# Autodesk Inventor assembly: VersaPlanetary One Stage 775
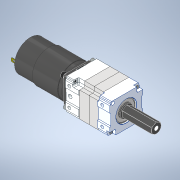
[picture p0: Inventor's stored thumbnail of the model, 180x180]
Saved by Autodesk Inventor 2022 (Build 260153000, 153)
## iProperties
Created: 2020-01-30
Part Number: VersaPlanetary One Stage 775
Document SubType Name: Assembly
Designer: aidan
Author: aidan
## Documents named in this file (10)
- C:\Users\Ty Gazaway\Documents\t3-cad\CAD\Generic and Stock\VersaPlanetary Parts\VersaPlanetary One Stage 775.iam
- C:\Users\Ty Gazaway\Documents\t3-cad\CAD\Generic and Stock\775 Pro.ipt
- C:\Users\Ty Gazaway\Documents\t3-cad\CAD\STEP Files\775_Series_Motor_Mounting_Plate.ipt
- C:\Users\Ty Gazaway\Documents\t3-cad\CAD\Generic and Stock\VersaPlanetary Parts\VersaPlanertary Mounting Block.ipt
- C:\Users\Ty Gazaway\Documents\t3-cad\CAD\Generic and Stock\VersaPlanetary Parts\VersaPlanetary Coupler.ipt
- C:\Users\Ty Gazaway\Documents\t3-cad\CAD\Generic and Stock\VersaPlanetary Parts\VersaPlanetary Motor Screw.ipt
- C:\Users\Ty Gazaway\Documents\t3-cad\CAD\Generic and Stock\VersaPlanetary Parts\VersaPlanetary Mounting Screw.ipt
- C:\Users\Ty Gazaway\Documents\t3-cad\CAD\Generic and Stock\VersaPlanetary Parts\VersaPlanetary Ring Gear.ipt
- C:\Users\Ty Gazaway\Documents\t3-cad\CAD\Generic and Stock\VersaPlanetary Parts\VersaPlanetary Long Screw.ipt
- C:\Users\Ty Gazaway\Documents\t3-cad\CAD\Generic and Stock\VersaPlanetary Parts\VersaPlanetary 0.500 Output.ipt
## Components (13 placed, 9 different names)
1. 775 Pro:1 — Mate:9, Mate:10, Mate:15, Flush:7, Mate:16, Mate:22
2. 775_Series_Motor_Mounting_Plate:1 — Mate:6, Mate:7, Mate:8, Mate:10, Mate:13, Mate:19, Flush:9
3. VersaPlanertary Mounting Block:1 — Flush:2, Mate:2, Mate:3, Mate:19, Mate:20, Mate:21, Mate:22, Flush:9, Mate:23, Mate:24, Mate:25
4. VersaPlanetary Coupler:1 — Mate:15, Flush:7
5. VersaPlanetary Motor Screw:1 — Mate:6, Flush:5, Mate:8, Mate:16
6. VersaPlanetary Motor Screw:2 — Mate:7, Flush:5, Mate:9
7. VersaPlanetary Mounting Screw:1 — Flush:6, Mate:21
8. VersaPlanetary Mounting Screw:2 — Flush:6, Mate:13, Mate:20
9. VersaPlanetary Ring Gear:1 — Flush:1, Flush:2, Flush:4, Mate:1, Mate:2, Mate:3
10. VersaPlanetary Ring Gear:2 — Flush:1, Flush:3, Flush:4, Mate:1, Mate:4, Mate:5
11. VersaPlanetary Long Screw:1 — Flush:8, Mate:25
12. VersaPlanetary Long Screw:2 — Flush:8, Mate:23, Mate:24
13. VersaPlanetary 0.500 Output:1 — Flush:3, Mate:4, Mate:5
## Relationships (29: Mate 20, Flush 9)
- Flush:1: VersaPlanetary Ring Gear:1 ↔ VersaPlanetary Ring Gear:2
- Flush:2: VersaPlanertary Mounting Block:1 ↔ VersaPlanetary Ring Gear:1
- Flush:3: VersaPlanetary Ring Gear:2 ↔ VersaPlanetary 0.500 Output:1
- Flush:4: VersaPlanetary Ring Gear:1 ↔ VersaPlanetary Ring Gear:2
- Mate:1: VersaPlanetary Ring Gear:1 ↔ VersaPlanetary Ring Gear:2
- Mate:2: VersaPlanertary Mounting Block:1 ↔ VersaPlanetary Ring Gear:1
- Mate:3: VersaPlanertary Mounting Block:1 ↔ VersaPlanetary Ring Gear:1
- Mate:4: VersaPlanetary Ring Gear:2 ↔ VersaPlanetary 0.500 Output:1
- Mate:5: VersaPlanetary Ring Gear:2 ↔ VersaPlanetary 0.500 Output:1
- Mate:6: 775_Series_Motor_Mounting_Plate:1 ↔ VersaPlanetary Motor Screw:1
- Mate:7: 775_Series_Motor_Mounting_Plate:1 ↔ VersaPlanetary Motor Screw:2
- Flush:5: VersaPlanetary Motor Screw:1 ↔ VersaPlanetary Motor Screw:2
- Mate:8: 775_Series_Motor_Mounting_Plate:1 ↔ VersaPlanetary Motor Screw:1
- Mate:9: 775 Pro:1 ↔ VersaPlanetary Motor Screw:2
- Mate:10: 775 Pro:1 ↔ 775_Series_Motor_Mounting_Plate:1
- Flush:6: VersaPlanetary Mounting Screw:1 ↔ VersaPlanetary Mounting Screw:2
- Mate:13: 775_Series_Motor_Mounting_Plate:1 ↔ VersaPlanetary Mounting Screw:2
- Mate:15: 775 Pro:1 ↔ VersaPlanetary Coupler:1
- Flush:7 (5.334 mm): 775 Pro:1 ↔ VersaPlanetary Coupler:1
- Mate:16: 775 Pro:1 ↔ VersaPlanetary Motor Screw:1
- Mate:19: 775_Series_Motor_Mounting_Plate:1 ↔ VersaPlanertary Mounting Block:1
- Flush:8: VersaPlanetary Long Screw:1 ↔ VersaPlanetary Long Screw:2
- Mate:20: VersaPlanertary Mounting Block:1 ↔ VersaPlanetary Mounting Screw:2
- Mate:21: VersaPlanertary Mounting Block:1 ↔ VersaPlanetary Mounting Screw:1
- Mate:22: 775 Pro:1 ↔ VersaPlanertary Mounting Block:1
- Flush:9: 775_Series_Motor_Mounting_Plate:1 ↔ VersaPlanertary Mounting Block:1
- Mate:23: VersaPlanertary Mounting Block:1 ↔ VersaPlanetary Long Screw:2
- Mate:24: VersaPlanertary Mounting Block:1 ↔ VersaPlanetary Long Screw:2
- Mate:25: VersaPlanertary Mounting Block:1 ↔ VersaPlanetary Long Screw:1
